# Autodesk Inventor assembly: DesignVer2
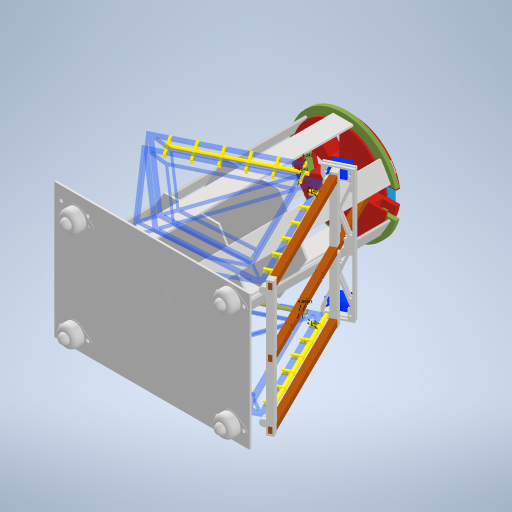
[picture p0: Inventor's stored thumbnail of the model, 512x512]
Saved by Autodesk Inventor 2024 (Build 280153000, 153)
## iProperties
Created: 2024-04-09
Part Number: DesignVer2
Document SubType Name: Assembly
Designer: USER
Author: USER
## Documents named in this file (15)
- E:\university\大三\大三下\機工實務\圖檔\DesignVer2\DesignVer2.iam
- E:\university\大三\大三下\機工實務\圖檔\DesignVer2\cow_wheel.ipt
- E:\university\大三\大三下\機工實務\圖檔\DesignVer2\back_down_hold.ipt
- E:\university\大三\大三下\機工實務\圖檔\DesignVer2\back_cir_hold.ipt
- E:\university\大三\大三下\機工實務\圖檔\DesignVer2\middle_space.ipt
- E:\university\大三\大三下\機工實務\圖檔\DesignVer2\rolling_plate.ipt
- E:\university\大三\大三下\機工實務\圖檔\DesignVer2\rolling_plate_top.ipt
- E:\university\大三\大三下\機工實務\圖檔\DesignVer2\rolling_plate_small.ipt
- E:\university\大三\大三下\機工實務\圖檔\DesignVer2\左右.ipt
- E:\university\大三\大三下\機工實務\圖檔\DesignVer2\左右2.ipt
- E:\university\大三\大三下\機工實務\圖檔\DesignVer2\馬達.ipt
- E:\university\大三\大三下\機工實務\圖檔\DesignVer2\軸.ipt
- E:\university\大三\大三下\機工實務\圖檔\DesignVer2\螺絲.ipt
- E:\university\大三\大三下\機工實務\圖檔\DesignVer2\sail.iam
- E:\university\大三\大三下\機工實務\圖檔\DesignVer2\Base_final.ipt
## Components (28 placed, 14 different names)
1. cow_wheel:1 — 貼合:82, 貼合:83, 貼合:84
2. cow_wheel:2 — 貼合:86
3. cow_wheel:3 — 貼合:80, 貼合:81, 貼合:85
4. cow_wheel:4 — 貼合:75, 貼合:76, 貼合:77, 貼合:78, 貼合:79
5. back_down_hold:1 — 貼合:99, 貼合:100, 貼合:101, 貼合:102
6. back_down_hold:2 — 貼合:34, 齊平:14, 相切:1, 齊平:28, 貼合:92, 貼合:93, 貼合:94
7. back_down_hold:3 — 齊平:5, 貼合:47, 齊平:13, 貼合:90, 貼合:91
8. back_down_hold:4 — 貼合:87, 貼合:97, 貼合:98
9. back_down_hold:5 — 齊平:6, 貼合:46, 齊平:12, 貼合:48, 貼合:88, 貼合:89, 貼合:105
10. back_down_hold:6 — 齊平:5, 齊平:6, 貼合:32, 貼合:33, 貼合:95, 貼合:96
11. back_cir_hold:1 — 貼合:32, 貼合:33, 貼合:34, 貼合:51, 貼合:103, 貼合:104, 角度:1
12. middle_space:1 — 齊平:13, 貼合:48, 齊平:14, 齊平:28
13. middle_space:2 — 貼合:46, 齊平:12, 貼合:47
14. rolling_plate:1 — 貼合:49, 貼合:50, 齊平:15, 貼合:51, 貼合:55, 齊平:22, 齊平:23
15. rolling_plate:2 — 貼合:56, 貼合:57, 齊平:24, 貼合:103, 貼合:104
16. rolling_plate_top:1 — 貼合:49, 貼合:50, 齊平:15, 相切:1, 貼合:58, 貼合:59, 貼合:60, 貼合:61, 貼合:62, 貼合:63, 角度:1
17. rolling_plate_small:1 — 貼合:52, 齊平:16, 齊平:19, 貼合:56, 齊平:24
18. rolling_plate_small:2 — 貼合:52, 貼合:53, 齊平:16, 齊平:17, 齊平:19, 齊平:20, 貼合:57
19. rolling_plate_small:3 — 貼合:53, 貼合:54, 齊平:17, 齊平:18, 齊平:20, 齊平:21
20. rolling_plate_small:4 — 貼合:54, 齊平:18, 齊平:21, 貼合:55, 齊平:22, 齊平:23
21. 左右:1 — 貼合:58, 貼合:59, 貼合:60, 貼合:66, 貼合:67, 齊平:26, 貼合:68, 齊平:27
22. 左右2:1 — 貼合:61, 貼合:62, 貼合:63, 貼合:74
23. 馬達:1 — 貼合:64, 貼合:65, 貼合:69, 貼合:70, 貼合:71
24. 軸:1 — 貼合:64, 貼合:65, 貼合:73, 貼合:106
25. 螺絲:1 — 齊平:25, 貼合:66, 貼合:67, 齊平:26, 貼合:69, 貼合:70
26. 螺絲:2 — 齊平:25, 貼合:68, 齊平:27, 貼合:71
27. sail:1 [sub-assembly] — 貼合:73, 貼合:74, 貼合:106
28. Base_final:1 — 貼合:75, 貼合:76, 貼合:77, 貼合:78, 貼合:79, 貼合:80, 貼合:81, 貼合:82, 貼合:83, 貼合:84, 貼合:85, 貼合:86, 貼合:87, 貼合:88, 貼合:89, 貼合:90, 貼合:91, 貼合:92, 貼合:93, 貼合:94, 貼合:95, 貼合:96, 貼合:97, 貼合:98, 貼合:99, 貼合:100, 貼合:101, 貼合:102, 貼合:105
## Relationships (84: Mate 63, Flush 19, Tangent 1, Angle 1)
- 齊平:5 [Flush]: back_down_hold:3 ↔ back_down_hold:6
- 齊平:6 [Flush]: back_down_hold:5 ↔ back_down_hold:6
- 貼合:32 [Mate]: back_down_hold:6 ↔ back_cir_hold:1
- 貼合:33 [Mate]: back_down_hold:6 ↔ back_cir_hold:1
- 貼合:34 [Mate]: back_down_hold:2 ↔ back_cir_hold:1
- 貼合:46 [Mate]: back_down_hold:5 ↔ middle_space:2
- 齊平:12 [Flush]: back_down_hold:5 ↔ middle_space:2
- 貼合:47 [Mate]: back_down_hold:3 ↔ middle_space:2
- 齊平:13 [Flush]: back_down_hold:3 ↔ middle_space:1
- 貼合:48 [Mate]: back_down_hold:5 ↔ middle_space:1
- 齊平:14 [Flush]: back_down_hold:2 ↔ middle_space:1
- 貼合:49 [Mate]: rolling_plate:1 ↔ rolling_plate_top:1
- 貼合:50 [Mate]: rolling_plate:1 ↔ rolling_plate_top:1
- 齊平:15 [Flush]: rolling_plate:1 ↔ rolling_plate_top:1
- 貼合:51 [Mate] (0.5 mm): back_cir_hold:1 ↔ rolling_plate:1
- 相切:1 [Tangent]: back_down_hold:2 ↔ rolling_plate_top:1
- 貼合:52 [Mate]: rolling_plate_small:1 ↔ rolling_plate_small:2
- 貼合:53 [Mate]: rolling_plate_small:2 ↔ rolling_plate_small:3
- 貼合:54 [Mate]: rolling_plate_small:3 ↔ rolling_plate_small:4
- 齊平:16 [Flush]: rolling_plate_small:1 ↔ rolling_plate_small:2
- 齊平:17 [Flush]: rolling_plate_small:2 ↔ rolling_plate_small:3
- 齊平:18 [Flush]: rolling_plate_small:3 ↔ rolling_plate_small:4
- 齊平:19 [Flush]: rolling_plate_small:1 ↔ rolling_plate_small:2
- 齊平:20 [Flush]: rolling_plate_small:2 ↔ rolling_plate_small:3
- 齊平:21 [Flush]: rolling_plate_small:3 ↔ rolling_plate_small:4
- 貼合:55 [Mate]: rolling_plate:1 ↔ rolling_plate_small:4
- 齊平:22 [Flush]: rolling_plate:1 ↔ rolling_plate_small:4
- 齊平:23 [Flush]: rolling_plate:1 ↔ rolling_plate_small:4
- 貼合:56 [Mate]: rolling_plate:2 ↔ rolling_plate_small:1
- 貼合:57 [Mate]: rolling_plate:2 ↔ rolling_plate_small:2
- 齊平:24 [Flush]: rolling_plate:2 ↔ rolling_plate_small:1
- 貼合:58 [Mate]: rolling_plate_top:1 ↔ 左右:1
- 貼合:59 [Mate]: rolling_plate_top:1 ↔ 左右:1
- 貼合:60 [Mate]: rolling_plate_top:1 ↔ 左右:1
- 貼合:61 [Mate]: rolling_plate_top:1 ↔ 左右2:1
- 貼合:62 [Mate]: rolling_plate_top:1 ↔ 左右2:1
- 貼合:63 [Mate]: rolling_plate_top:1 ↔ 左右2:1
- 貼合:64 [Mate]: 馬達:1 ↔ 軸:1
- 貼合:65 [Mate]: 馬達:1 ↔ 軸:1
- 齊平:25 [Flush]: 螺絲:1 ↔ 螺絲:2
- 貼合:66 [Mate]: 左右:1 ↔ 螺絲:1
- 貼合:67 [Mate]: 左右:1 ↔ 螺絲:1
- 齊平:26 [Flush]: 左右:1 ↔ 螺絲:1
- 貼合:68 [Mate]: 左右:1 ↔ 螺絲:2
- 齊平:27 [Flush]: 左右:1 ↔ 螺絲:2
- 貼合:69 [Mate]: 馬達:1 ↔ 螺絲:1
- 貼合:70 [Mate]: 馬達:1 ↔ 螺絲:1
- 貼合:71 [Mate]: 馬達:1 ↔ 螺絲:2
- 齊平:28 [Flush]: back_down_hold:2 ↔ middle_space:1
- 貼合:73 [Mate]: 軸:1 ↔ sail:1
- 貼合:74 [Mate] (0.1 mm): 左右2:1 ↔ sail:1
- 貼合:75 [Mate]: cow_wheel:4 ↔ Base_final:1
- 貼合:76 [Mate]: cow_wheel:4 ↔ Base_final:1
- 貼合:77 [Mate]: cow_wheel:4 ↔ Base_final:1
- 貼合:78 [Mate]: cow_wheel:4 ↔ Base_final:1
- 貼合:79 [Mate]: cow_wheel:4 ↔ Base_final:1
- 貼合:80 [Mate]: cow_wheel:3 ↔ Base_final:1
- 貼合:81 [Mate]: cow_wheel:3 ↔ Base_final:1
- 貼合:82 [Mate]: cow_wheel:1 ↔ Base_final:1
- 貼合:83 [Mate]: cow_wheel:1 ↔ Base_final:1
- 貼合:84 [Mate]: cow_wheel:1 ↔ Base_final:1
- 貼合:85 [Mate]: cow_wheel:3 ↔ Base_final:1
- 貼合:86 [Mate]: cow_wheel:2 ↔ Base_final:1
- 貼合:87 [Mate]: back_down_hold:4 ↔ Base_final:1
- 貼合:88 [Mate]: back_down_hold:5 ↔ Base_final:1
- 貼合:89 [Mate]: back_down_hold:5 ↔ Base_final:1
- 貼合:90 [Mate]: back_down_hold:3 ↔ Base_final:1
- 貼合:91 [Mate]: back_down_hold:3 ↔ Base_final:1
- 貼合:92 [Mate]: back_down_hold:2 ↔ Base_final:1
- 貼合:93 [Mate]: back_down_hold:2 ↔ Base_final:1
- 貼合:94 [Mate]: back_down_hold:2 ↔ Base_final:1
- 貼合:95 [Mate]: back_down_hold:6 ↔ Base_final:1
- 貼合:96 [Mate]: back_down_hold:6 ↔ Base_final:1
- 貼合:97 [Mate]: back_down_hold:4 ↔ Base_final:1
- 貼合:98 [Mate]: back_down_hold:4 ↔ Base_final:1
- 貼合:99 [Mate]: back_down_hold:1 ↔ Base_final:1
- 貼合:100 [Mate]: back_down_hold:1 ↔ Base_final:1
- 貼合:101 [Mate]: back_down_hold:1 ↔ Base_final:1
- 貼合:102 [Mate]: back_down_hold:1 ↔ Base_final:1
- 貼合:103 [Mate] (0.5 mm): back_cir_hold:1 ↔ rolling_plate:2
- 貼合:104 [Mate]: back_cir_hold:1 ↔ rolling_plate:2
- 貼合:105 [Mate]: back_down_hold:5 ↔ Base_final:1
- 貼合:106 [Mate]: 軸:1 ↔ sail:1
- 角度:1 [Angle] (0 deg): back_cir_hold:1 ↔ rolling_plate_top:1
